# Autodesk Inventor assembly: Assey_Course_C_v1
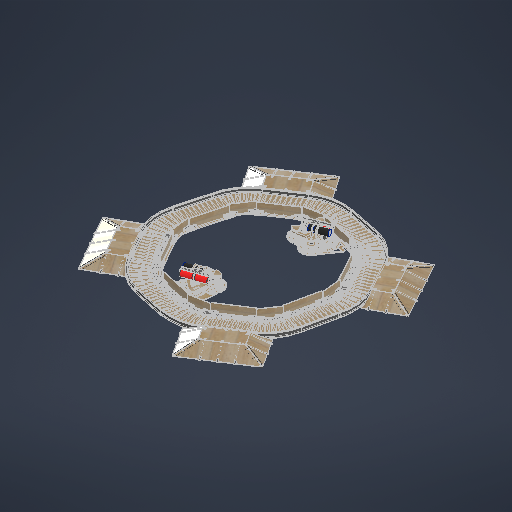
[picture p0: Inventor's stored thumbnail of the model, 512x512]
Saved by Autodesk Inventor 2027.1 (Build 311270010, 270A)
## iProperties
Created: 2026-08-08
Part Number: Assey_Course_C_v1
Document SubType Name: Assembly
Designer: takuya
Author: takuya
## Documents named in this file (4)
- C:\Users\takuya\Documents\D2_conveyor\Assey_Course_C.iam
- C:\Users\takuya\Documents\D2_conveyor\power_module\Assy_power_module.iam
- C:\Users\takuya\Documents\D2_conveyor\Assely_Curve_Liner_Slope.iam
- C:\Users\takuya\Documents\D2_conveyor\liniar_module\Assy_linear_module.iam
## Components (11 placed, 3 different names)
1. Assy_power_module:2 [sub-assembly]
2. Assy_power_module:3 [sub-assembly] — メイト:1, メイト:2, メイト:3
3. Assy_power_module:4 [sub-assembly] — メイト:4, メイト:5, メイト:6
4. Assely_Curve_Liner_Slope:1 [sub-assembly] — 回転:5, 回転:6
5. Assy_linear_module:1 [sub-assembly] — メイト:1, メイト:2, メイト:3, 回転:1, メイト:7, 角度:1
6. Assy_linear_module:2 [sub-assembly] — メイト:4, メイト:5, メイト:6, 回転:4, 回転:5, 角度:4
7. Assely_Curve_Liner_Slope:2 [sub-assembly] — 回転:7, メイト:7, 角度:1, 角度:2
8. Assy_linear_module:3 [sub-assembly] — 回転:6, 回転:7, 角度:2
9. Assely_Curve_Liner_Slope:3 [sub-assembly] — 回転:3, 回転:4, 角度:4
10. Assy_linear_module:4 [sub-assembly] — 回転:2, 回転:3, 角度:3
11. Assely_Curve_Liner_Slope:4 [sub-assembly] — 回転:1, 回転:2, 角度:3
## Relationships (18: Mate 7, RevoluteJoint 7, Angle 4)
- メイト:1 [Mate]: Assy_power_module:3 ↔ Assy_linear_module:1
- メイト:2 [Mate]: Assy_power_module:3 ↔ Assy_linear_module:1
- メイト:3 [Mate]: Assy_power_module:3 ↔ Assy_linear_module:1
- メイト:4 [Mate]: Assy_power_module:4 ↔ Assy_linear_module:2
- メイト:5 [Mate]: Assy_power_module:4 ↔ Assy_linear_module:2
- メイト:6 [Mate]: Assy_power_module:4 ↔ Assy_linear_module:2
- 回転:1 [RevoluteJoint]: Assy_linear_module:1 ↔ Assely_Curve_Liner_Slope:4
- 回転:2 [RevoluteJoint]: Assy_linear_module:4 ↔ Assely_Curve_Liner_Slope:4
- 回転:3 [RevoluteJoint]: Assely_Curve_Liner_Slope:3 ↔ Assy_linear_module:4
- 回転:4 [RevoluteJoint]: Assy_linear_module:2 ↔ Assely_Curve_Liner_Slope:3
- 回転:5 [RevoluteJoint]: Assely_Curve_Liner_Slope:1 ↔ Assy_linear_module:2
- 回転:6 [RevoluteJoint]: Assely_Curve_Liner_Slope:1 ↔ Assy_linear_module:3
- 回転:7 [RevoluteJoint]: Assely_Curve_Liner_Slope:2 ↔ Assy_linear_module:3
- メイト:7 [Mate]: Assy_linear_module:1 ↔ Assely_Curve_Liner_Slope:2
- 角度:1 [Angle] (180 deg): Assy_linear_module:1 ↔ Assely_Curve_Liner_Slope:2
- 角度:2 [Angle] (180 deg): Assely_Curve_Liner_Slope:2 ↔ Assy_linear_module:3
- 角度:3 [Angle] (180 deg): Assy_linear_module:4 ↔ Assely_Curve_Liner_Slope:4
- 角度:4 [Angle] (180 deg): Assy_linear_module:2 ↔ Assely_Curve_Liner_Slope:3
